# Autodesk Inventor assembly: Baugruppe1
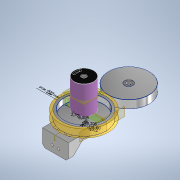
[picture p0: Inventor's stored thumbnail of the model, 180x180]
Saved by Autodesk Inventor 2022 (Build 260153000, 153)
## iProperties
Created: 2022-11-23
Part Number: Baugruppe1
Document SubType Name: Assembly
Designer: Friedrich Walmrath
Author: Friedrich Walmrath
## Documents named in this file (8)
- E:\Kartenzar70\Kartenzar70\CAD-Dateien\Abschusseinheit\v1\testaufbau\Baugruppe1.iam
- E:\Kartenzar70\Kartenzar70\CAD-Dateien\Abschusseinheit\simtest\Baugruppe1.iam
- E:\Kartenzar70\Kartenzar70\CAD-Dateien\Abschusseinheit\v1\gegenroller.ipt
- E:\Kartenzar70\Kartenzar70\CAD-Dateien\Abschusseinheit\v1\motor.ipt
- C:\Users\fritz\Documents\Inventor\Content Center Files\R2022\de-DE\ISO 4026\ISO 4026 - M2 x 2,5 - ISO.ipt
- E:\Kartenzar70\Kartenzar70\CAD-Dateien\Abschusseinheit\v1\mr106 lager dummy.ipt
- E:\Kartenzar70\Kartenzar70\CAD-Dateien\Abschusseinheit\v1\testaufbau\halter1.ipt
- E:\Kartenzar70\Kartenzar70\CAD-Dateien\Abschusseinheit\v1\testaufbau\halter1_2.ipt
## Components (9 placed, 7 different names)
1. Baugruppe1:1 [sub-assembly] — Winkel:1, Tangential:1, Passend:1, Passend:2, Passend:3, Fluchtend:1, Passend:6, Passend:7
2. gegenroller:1 — Winkel:1, Tangential:1, Passend:5, Fluchtend:1, Passend:8, Passend:9, Passend:10, Passend:11, Passend:14
3. motor:1 — Passend:1, Passend:2, Passend:4
4. ISO 4026 M2 x 2,5:1 — Passend:3, Passend:4
5. mr106 lager dummy:1 — Passend:10, Passend:11
6. mr106 lager dummy:2 — Passend:8, Passend:9
7. mr106 lager dummy:3 — Passend:6, Passend:7, Passend:12, Passend:13, Passend:15
8. halter1:1 — Passend:12, Passend:13, Passend:14, Passend:16
9. halter1_2:1 — Passend:15, Passend:16
## Relationships (19: Mate 16, Angle 1, Tangent 1, Flush 1)
- Winkel:1 [Angle] (0 deg): Baugruppe1:1 ↔ gegenroller:1
- Tangential:1: Baugruppe1:1 ↔ gegenroller:1
- Passend:1 [Mate]: Baugruppe1:1 ↔ motor:1
- Passend:2 [Mate]: Baugruppe1:1 ↔ motor:1
- Passend:3 [Mate]: Baugruppe1:1 ↔ ISO 4026 M2 x 2,5:1
- Passend:4 [Mate]: motor:1 ↔ ISO 4026 M2 x 2,5:1
- Passend:5 [Mate]: gegenroller:1
- Fluchtend:1 [Flush]: Baugruppe1:1 ↔ gegenroller:1
- Passend:6 [Mate]: Baugruppe1:1 ↔ mr106 lager dummy:3
- Passend:7 [Mate]: Baugruppe1:1 ↔ mr106 lager dummy:3
- Passend:8 [Mate]: gegenroller:1 ↔ mr106 lager dummy:2
- Passend:9 [Mate]: gegenroller:1 ↔ mr106 lager dummy:2
- Passend:10 [Mate]: gegenroller:1 ↔ mr106 lager dummy:1
- Passend:11 [Mate]: gegenroller:1 ↔ mr106 lager dummy:1
- Passend:12 [Mate]: mr106 lager dummy:3 ↔ halter1:1
- Passend:13 [Mate]: mr106 lager dummy:3 ↔ halter1:1
- Passend:14 [Mate]: gegenroller:1 ↔ halter1:1
- Passend:15 [Mate]: mr106 lager dummy:3 ↔ halter1_2:1
- Passend:16 [Mate]: halter1:1 ↔ halter1_2:1
